# Autodesk Inventor assembly: Main_Bot
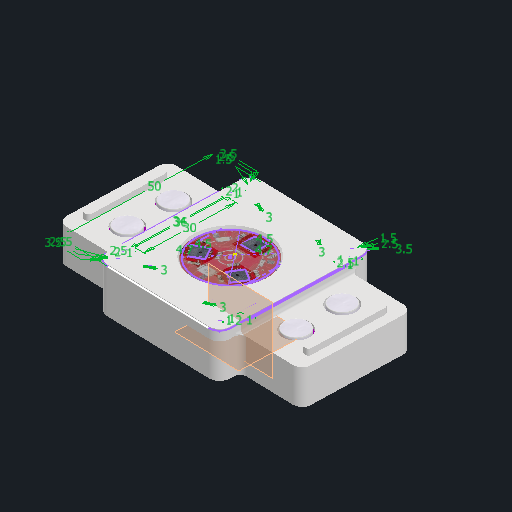
[picture p0: Inventor's stored thumbnail of the model, 512x512]
Saved by Autodesk Inventor 2026 (Build 300175000, 175)
## iProperties
Created: 2025-04-14
Part Number: Main_Bot
Document SubType Name: Assembly
Designer: ct_vi
Author: ct_vi
## Documents named in this file (5)
- C:\Users\ct_vi\Documents\Capstone_Research_3D_Files\Main_Bot.iam
- C:\Users\ct_vi\Documents\Capstone_Research_3D_Files\Spectral_Sensor.ipt
- C:\Users\ct_vi\Documents\Capstone_Research_3D_Files\Spectral_Case_Angled.ipt
- C:\Users\ct_vi\Documents\Capstone_Research_3D_Files\Gas_Sensorsipt.ipt
- C:\Users\ct_vi\Documents\Capstone_Research_3D_Files\4Pin_Set.iam
## Components (10 placed, 4 different names)
1. Spectral_Sensor:1 — Mate:1, Mate:2, Mate:11
2. Spectral_Case_Bot:1 — Mate:1, Mate:2, Mate:11, Mate:13, Mate:14, Mate:15, Mate:20, Mate:21, Mate:22, Mate:23, Mate:24, Mate:25, Mate:26, Mate:27
3. Gas_Sensorsipt:1 — Mate:12, Flush:1, Flush:2, Mate:13, Mate:14, Mate:15
4. 4Pin_Set:1 [sub-assembly] — Mate:12, Flush:1, Flush:2
5. Gas_Sensorsipt:2 — Mate:22, Mate:23, Mate:24
6. 4Pin_Set:2 [sub-assembly]
7. Gas_Sensorsipt:3 — Mate:20, Mate:21
8. 4Pin_Set:3 [sub-assembly]
9. Gas_Sensorsipt:5 — Mate:25, Mate:26, Mate:27
10. 4Pin_Set:5 [sub-assembly]
## Relationships (26: Mate 18, Flush 8)
- Mate:1: Spectral_Sensor:1 ↔ Spectral_Case_Bot:1
- Mate:2: Spectral_Sensor:1 ↔ Spectral_Case_Bot:1
- Mate:11: Spectral_Sensor:1 ↔ Spectral_Case_Bot:1
- Mate:12: Gas_Sensorsipt:1 ↔ 4Pin_Set:1
- Flush:1 (-1.68 mm): Gas_Sensorsipt:1 ↔ 4Pin_Set:1
- Flush:2 (1.25 mm): Gas_Sensorsipt:1 ↔ 4Pin_Set:1
- Mate:13: Spectral_Case_Bot:1 ↔ Gas_Sensorsipt:1
- Mate:14: Spectral_Case_Bot:1 ↔ Gas_Sensorsipt:1
- Mate:15: Spectral_Case_Bot:1 ↔ Gas_Sensorsipt:1
- [Mate]: Gas_Sensorsipt:2 ↔ 4Pin_Set:2
- [Flush] (-1.68 mm): Gas_Sensorsipt:2 ↔ 4Pin_Set:2
- [Flush] (1.25 mm): Gas_Sensorsipt:2 ↔ 4Pin_Set:2
- [Mate]: Gas_Sensorsipt:3 ↔ 4Pin_Set:3
- [Flush] (-1.68 mm): Gas_Sensorsipt:3 ↔ 4Pin_Set:3
- [Flush] (1.25 mm): Gas_Sensorsipt:3 ↔ 4Pin_Set:3
- [Mate]: Gas_Sensorsipt:5 ↔ 4Pin_Set:5
- [Flush] (-1.68 mm): Gas_Sensorsipt:5 ↔ 4Pin_Set:5
- [Flush] (1.25 mm): Gas_Sensorsipt:5 ↔ 4Pin_Set:5
- Mate:20: Spectral_Case_Bot:1 ↔ Gas_Sensorsipt:3
- Mate:21: Spectral_Case_Bot:1 ↔ Gas_Sensorsipt:3
- Mate:22: Spectral_Case_Bot:1 ↔ Gas_Sensorsipt:2
- Mate:23: Spectral_Case_Bot:1 ↔ Gas_Sensorsipt:2
- Mate:24: Spectral_Case_Bot:1 ↔ Gas_Sensorsipt:2
- Mate:25: Spectral_Case_Bot:1 ↔ Gas_Sensorsipt:5
- Mate:26: Spectral_Case_Bot:1 ↔ Gas_Sensorsipt:5
- Mate:27: Spectral_Case_Bot:1 ↔ Gas_Sensorsipt:5
## Named parameters: d40_d33 = 0 mm, d41_d35 = -1.68 mm, d42_d36 = 1.25 mm, d43_d33 = 0 mm, d44_d35 = -1.68 mm, d45_d36 = 1.25 mm, d49_d33 = 0 mm, d50_d35 = -1.68 mm, d51_d36 = 1.25 mm
